# Autodesk Inventor assembly: Rover
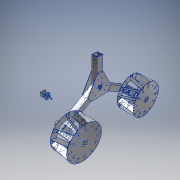
[picture p0: Inventor's stored thumbnail of the model, 180x180]
Saved by Autodesk Inventor 2019 (Build 230136000, 136)
## iProperties
Created: 2018-10-14
Part Number: Rover
Document SubType Name: Assembly
Designer: Adhik
Author: Adhik
## Documents named in this file (7)
- E:\CAD\Julie\Rover.iam
- E:\CAD\Julie\Outer Gusset Plate.ipt
- E:\CAD\Julie\Drive Arm.iam
- E:\CAD\Julie\Arm 8 inch.ipt
- E:\CAD\Julie\Arm Bearing.ipt
- E:\CAD\Julie\Gearbox.ipt
- E:\CAD\Julie\Gearbox Shaft.ipt
## Components (11 placed, 6 different names)
1. Outer Gusset Plate:1 — Flush:1, Flush:2, Mate:1, Mate:2, Mate:3, Mate:4, Mate:5, Mate:6, Mate:8, Mate:9, Mate:10, Insert:2
2. Outer Gusset Plate:2 — Flush:1, Flush:2, Mate:7, Insert:1
3. Drive Arm:1 [sub-assembly] — Mate:1, Mate:3, Mate:4, Mate:7, Mate:11, Mate:12, Mate:13
4. Drive Arm:2 [sub-assembly] — Mate:2, Mate:5, Mate:6
5. Arm 8 inch:1 — Mate:8, Mate:9, Mate:10
6. Arm Bearing:1 — Insert:2
7. Arm Bearing:2 — Insert:1
8. Gearbox:1 — Insert:3
9. Gearbox:2 — Insert:4, Mate:11, Mate:12, Mate:13
10. Gearbox Shaft:1 — Insert:3
11. Gearbox Shaft:2 — Insert:4
## Relationships (19: Mate 13, Insert 4, Flush 2)
- Flush:1: Outer Gusset Plate:1 ↔ Outer Gusset Plate:2
- Flush:2: Outer Gusset Plate:1 ↔ Outer Gusset Plate:2
- Mate:1: Outer Gusset Plate:1 ↔ Drive Arm:1
- Mate:2: Outer Gusset Plate:1 ↔ Drive Arm:2
- Mate:3: Outer Gusset Plate:1 ↔ Drive Arm:1
- Mate:4: Outer Gusset Plate:1 ↔ Drive Arm:1
- Mate:5: Outer Gusset Plate:1 ↔ Drive Arm:2
- Mate:6: Outer Gusset Plate:1 ↔ Drive Arm:2
- Mate:7: Outer Gusset Plate:2 ↔ Drive Arm:1
- Mate:8: Outer Gusset Plate:1 ↔ Arm 8 inch:1
- Mate:9: Outer Gusset Plate:1 ↔ Arm 8 inch:1
- Mate:10: Outer Gusset Plate:1 ↔ Arm 8 inch:1
- Insert:1: Outer Gusset Plate:2 ↔ Arm Bearing:2
- Insert:2: Outer Gusset Plate:1 ↔ Arm Bearing:1
- Insert:3: Gearbox:1 ↔ Gearbox Shaft:1
- Insert:4: Gearbox:2 ↔ Gearbox Shaft:2
- Mate:11: Drive Arm:1 ↔ Gearbox:2
- Mate:12: Drive Arm:1 ↔ Gearbox:2
- Mate:13: Drive Arm:1 ↔ Gearbox:2
